# Autodesk Inventor assembly: Drone Assembly
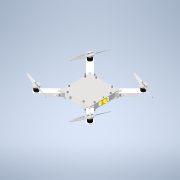
[picture p0: Inventor's stored thumbnail of the model, 180x180]
Saved by Autodesk Inventor 2021 (Build 250183000, 183)
## iProperties
Created: 2020-11-19
Part Number: Drone Assembly
Document SubType Name: Assembly
Designer: Pysion
Author: Pysion
## Documents named in this file (10)
- C:\Users\Pysion\Documents\GrabCAD\V1\Drone Assembly.iam
- C:\Users\Pysion\Documents\GrabCAD\V1\ArmAssembly.iam
- C:\Users\Pysion\Documents\GrabCAD\V1\Battery Pack.ipt
- C:\Users\Pysion\Documents\GrabCAD\V1\bottom_plate.ipt
- C:\Users\Pysion\Documents\GrabCAD\V1\charging_port.ipt
- C:\Users\Pysion\Documents\GrabCAD\V1\Electronics.ipt
- C:\Users\Pysion\Documents\GrabCAD\V1\top_plate.ipt
- C:\Users\Pysion\Documents\GrabCAD\V1\ContentCenter\en-US\AS 1420\AS 1420 - 1973 - M6 x 20.ipt
- C:\Users\Pysion\Documents\GrabCAD\V1\ContentCenter\en-US\AS 1420\AS 1420 - 1973 - M5 x 14.ipt
- C:\Users\Pysion\Documents\GrabCAD\V1\ContentCenter\en-US\AS 1420\AS 1420 - 1973 - M4 x 10.ipt
## Components (36 placed, 9 different names)
1. Battery Pack:1 — Mate:11, Flush:3, Flush:5
2. bottom_plate:1 — Flush:2, Mate:11, Flush:3, Flush:4, Mate:12, Flush:5, Flush:6, Flush:7, Mate:69, Mate:70, Mate:71, Mate:72, Flush:8, Flush:9, Flush:10, Flush:11, Flush:12, Flush:13, Flush:14, Flush:15, Flush:16, Insert:9, Insert:10, Insert:11, Insert:12, Insert:13, Insert:14, Insert:15, Insert:16, Insert:17, Insert:18, Insert:19, Insert:20, Insert:21, Insert:22, Insert:23, Insert:24, Angle:16, Insert:26, Insert:27, Angle:19
3. charging_port:1 — Flush:2, Flush:7, Mate:74
4. Electronics:1 — Flush:4, Mate:12, Flush:6
5. top_plate:1 — Mate:73, Flush:17, Flush:18, Flush:19, Insert:1, Insert:2, Insert:3, Insert:4, Insert:5, Insert:6, Insert:7, Insert:8, Insert:25, Mate:74
6. ArmAssembly:5 [sub-assembly] — Mate:70, Flush:10, Flush:11
7. ArmAssembly:6 [sub-assembly] — Mate:69, Flush:8, Flush:9, Flush:16, Flush:18, Flush:19
8. ArmAssembly:7 [sub-assembly] — Mate:71, Flush:14, Flush:15, Mate:73, Flush:17
9. ArmAssembly:8 [sub-assembly] — Mate:72, Flush:12, Flush:13
10. AS 1420 - Metric M6 x 20:2 — Insert:5
11. AS 1420 - Metric M6 x 20:1 — Insert:1
12. AS 1420 - Metric M6 x 20:3 — Insert:8
13. AS 1420 - Metric M6 x 20:4 — Insert:6
14. AS 1420 - Metric M6 x 20:5 — Insert:4
15. AS 1420 - Metric M6 x 20:6 — Insert:2
16. AS 1420 - Metric M6 x 20:7 — Insert:7
17. AS 1420 - Metric M6 x 20:8 — Insert:3
18. AS 1420 - Metric M4 x 10:1 — Insert:26, Angle:17, Angle:18
19. AS 1420 - Metric M4 x 10:2 — Insert:25, Angle:17
20. AS 1420 - Metric M4 x 10:3 — Insert:27, Angle:18, Angle:19
21. AS 1420 - Metric M5 x 14:1 — Insert:9, Angle:1
22. AS 1420 - Metric M5 x 14:2 — Insert:11, Angle:15, Angle:16
23. AS 1420 - Metric M5 x 14:3 — Insert:10, Angle:1, Angle:2
24. AS 1420 - Metric M5 x 14:4 — Insert:12, Angle:14, Angle:15
25. AS 1420 - Metric M5 x 14:5 — Insert:21, Angle:4, Angle:6
26. AS 1420 - Metric M5 x 14:6 — Insert:22, Angle:4, Angle:5
27. AS 1420 - Metric M5 x 14:7 — Insert:23, Angle:2, Angle:3
28. AS 1420 - Metric M5 x 14:8 — Insert:24, Angle:3, Angle:5
29. AS 1420 - Metric M5 x 14:9 — Insert:16, Angle:10, Angle:11
30. AS 1420 - Metric M5 x 14:10 — Insert:15, Angle:11, Angle:12
31. AS 1420 - Metric M5 x 14:11 — Insert:13, Angle:13, Angle:14
32. AS 1420 - Metric M5 x 14:12 — Insert:14, Angle:12, Angle:13
33. AS 1420 - Metric M5 x 14:13 — Insert:19, Angle:7, Angle:8
34. AS 1420 - Metric M5 x 14:14 — Insert:17, Angle:9, Angle:10
35. AS 1420 - Metric M5 x 14:15 — Insert:18, Angle:8, Angle:9
36. AS 1420 - Metric M5 x 14:16 — Insert:20, Angle:6, Angle:7
## Relationships (72: Insert 27, Angle 19, Flush 18, Mate 8)
- Flush:2 (80 mm): bottom_plate:1 ↔ charging_port:1
- Mate:11: Battery Pack:1 ↔ bottom_plate:1
- Flush:3 (50 mm): Battery Pack:1 ↔ bottom_plate:1
- Flush:4 (50 mm): bottom_plate:1 ↔ Electronics:1
- Mate:12: bottom_plate:1 ↔ Electronics:1
- Flush:5 (50 mm): Battery Pack:1 ↔ bottom_plate:1
- Flush:6 (110 mm): bottom_plate:1 ↔ Electronics:1
- Flush:7: bottom_plate:1 ↔ charging_port:1
- Mate:69: bottom_plate:1 ↔ ArmAssembly:6
- Mate:70: bottom_plate:1 ↔ ArmAssembly:5
- Mate:71: bottom_plate:1 ↔ ArmAssembly:7
- Mate:72: bottom_plate:1 ↔ ArmAssembly:8
- Flush:8: bottom_plate:1 ↔ ArmAssembly:6
- Flush:9: bottom_plate:1 ↔ ArmAssembly:6
- Flush:10: bottom_plate:1 ↔ ArmAssembly:5
- Flush:11: bottom_plate:1 ↔ ArmAssembly:5
- Flush:12: bottom_plate:1 ↔ ArmAssembly:8
- Flush:13: bottom_plate:1 ↔ ArmAssembly:8
- Flush:14: bottom_plate:1 ↔ ArmAssembly:7
- Flush:15: bottom_plate:1 ↔ ArmAssembly:7
- Flush:16: bottom_plate:1 ↔ ArmAssembly:6
- Mate:73: top_plate:1 ↔ ArmAssembly:7
- Flush:17: top_plate:1 ↔ ArmAssembly:7
- Flush:18: top_plate:1 ↔ ArmAssembly:6
- Flush:19: top_plate:1 ↔ ArmAssembly:6
- Insert:1: top_plate:1 ↔ AS 1420 - Metric M6 x 20:1
- Insert:2: top_plate:1 ↔ AS 1420 - Metric M6 x 20:6
- Insert:3: top_plate:1 ↔ AS 1420 - Metric M6 x 20:8
- Insert:4: top_plate:1 ↔ AS 1420 - Metric M6 x 20:5
- Insert:5: top_plate:1 ↔ AS 1420 - Metric M6 x 20:2
- Insert:6: top_plate:1 ↔ AS 1420 - Metric M6 x 20:4
- Insert:7: top_plate:1 ↔ AS 1420 - Metric M6 x 20:7
- Insert:8: top_plate:1 ↔ AS 1420 - Metric M6 x 20:3
- Insert:9: bottom_plate:1 ↔ AS 1420 - Metric M5 x 14:1
- Insert:10: bottom_plate:1 ↔ AS 1420 - Metric M5 x 14:3
- Insert:11: bottom_plate:1 ↔ AS 1420 - Metric M5 x 14:2
- Insert:12: bottom_plate:1 ↔ AS 1420 - Metric M5 x 14:4
- Insert:13: bottom_plate:1 ↔ AS 1420 - Metric M5 x 14:11
- Insert:14: bottom_plate:1 ↔ AS 1420 - Metric M5 x 14:12
- Insert:15: bottom_plate:1 ↔ AS 1420 - Metric M5 x 14:10
- Insert:16: bottom_plate:1 ↔ AS 1420 - Metric M5 x 14:9
- Insert:17: bottom_plate:1 ↔ AS 1420 - Metric M5 x 14:14
- Insert:18: bottom_plate:1 ↔ AS 1420 - Metric M5 x 14:15
- Insert:19: bottom_plate:1 ↔ AS 1420 - Metric M5 x 14:13
- Insert:20: bottom_plate:1 ↔ AS 1420 - Metric M5 x 14:16
- Insert:21: bottom_plate:1 ↔ AS 1420 - Metric M5 x 14:5
- Insert:22: bottom_plate:1 ↔ AS 1420 - Metric M5 x 14:6
- Insert:23: bottom_plate:1 ↔ AS 1420 - Metric M5 x 14:7
- Insert:24: bottom_plate:1 ↔ AS 1420 - Metric M5 x 14:8
- Angle:1 (0 deg): AS 1420 - Metric M5 x 14:1 ↔ AS 1420 - Metric M5 x 14:3
- Angle:2 (0 deg): AS 1420 - Metric M5 x 14:3 ↔ AS 1420 - Metric M5 x 14:7
- Angle:3 (0 deg): AS 1420 - Metric M5 x 14:7 ↔ AS 1420 - Metric M5 x 14:8
- Angle:4 (0 deg): AS 1420 - Metric M5 x 14:5 ↔ AS 1420 - Metric M5 x 14:6
- Angle:5 (0 deg): AS 1420 - Metric M5 x 14:6 ↔ AS 1420 - Metric M5 x 14:8
- Angle:6 (0 deg): AS 1420 - Metric M5 x 14:5 ↔ AS 1420 - Metric M5 x 14:16
- Angle:7 (0 deg): AS 1420 - Metric M5 x 14:13 ↔ AS 1420 - Metric M5 x 14:16
- Angle:8 (0 deg): AS 1420 - Metric M5 x 14:13 ↔ AS 1420 - Metric M5 x 14:15
- Angle:9 (0 deg): AS 1420 - Metric M5 x 14:14 ↔ AS 1420 - Metric M5 x 14:15
- Angle:10 (0 deg): AS 1420 - Metric M5 x 14:9 ↔ AS 1420 - Metric M5 x 14:14
- Angle:11 (0 deg): AS 1420 - Metric M5 x 14:9 ↔ AS 1420 - Metric M5 x 14:10
- Angle:12 (0 deg): AS 1420 - Metric M5 x 14:10 ↔ AS 1420 - Metric M5 x 14:12
- Angle:13 (0 deg): AS 1420 - Metric M5 x 14:11 ↔ AS 1420 - Metric M5 x 14:12
- Angle:14 (0 deg): AS 1420 - Metric M5 x 14:4 ↔ AS 1420 - Metric M5 x 14:11
- Angle:15 (0 deg): AS 1420 - Metric M5 x 14:2 ↔ AS 1420 - Metric M5 x 14:4
- Angle:16 (0 deg): bottom_plate:1 ↔ AS 1420 - Metric M5 x 14:2
- Insert:25: top_plate:1 ↔ AS 1420 - Metric M4 x 10:2
- Insert:26: bottom_plate:1 ↔ AS 1420 - Metric M4 x 10:1
- Insert:27: bottom_plate:1 ↔ AS 1420 - Metric M4 x 10:3
- Angle:17 (0 deg): AS 1420 - Metric M4 x 10:1 ↔ AS 1420 - Metric M4 x 10:2
- Angle:18 (0 deg): AS 1420 - Metric M4 x 10:1 ↔ AS 1420 - Metric M4 x 10:3
- Angle:19 (0 deg): bottom_plate:1 ↔ AS 1420 - Metric M4 x 10:3
- Mate:74: charging_port:1 ↔ top_plate:1
